# Autodesk Inventor assembly: cradleAssembly
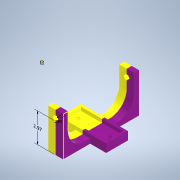
[picture p0: Inventor's stored thumbnail of the model, 180x180]
Saved by Autodesk Inventor 2022 (Build 260153070, 153G)
## iProperties
Created: 2021-06-29
Part Number: cradleAssembly
Document SubType Name: Assembly
Designer: robst
Author: robst
## Documents named in this file (3)
- C:\git\CAD-Development\robSteele\ShapeWays\TelescopeProjects\TelescopeMountNov2020\cradleAssembly.iam
- C:\git\CAD-Development\robSteele\ShapeWays\TelescopeProjects\TelescopeMountNov2020\connectorToTubeBrackeCradlePrintBack.ipt
- C:\git\CAD-Development\robSteele\ShapeWays\TelescopeProjects\TelescopeMountNov2020\connectorToTubeBrackeCradlePrintFront.ipt
## Components (2 placed, 2 different names)
1. connectorToTubeBrackeCradlePrintBack:1 — Mate:1, Flush:1, Flush:2
2. connectorToTubeBrackeCradlePrintFront:1 — Mate:1, Flush:1, Flush:2
## Relationships (3: Flush 2, Mate 1)
- Mate:1: connectorToTubeBrackeCradlePrintBack:1 ↔ connectorToTubeBrackeCradlePrintFront:1
- Flush:1: connectorToTubeBrackeCradlePrintBack:1 ↔ connectorToTubeBrackeCradlePrintFront:1
- Flush:2: connectorToTubeBrackeCradlePrintBack:1 ↔ connectorToTubeBrackeCradlePrintFront:1
